# Autodesk Inventor assembly: servoAssembly
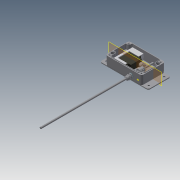
[picture p0: Inventor's stored thumbnail of the model, 180x180]
Saved by Autodesk Inventor 2018 (Build 220112000, 112)
## iProperties
Created: 2020-02-20
Part Number: servoAssembly
Document SubType Name: Assembly
Designer: anirudh
Author: anirudh
## Documents named in this file (10)
- D:\Silicon Sharks\2019-2020\servoBox\servoAssembly.iam
- D:\Silicon Sharks\2019-2020\servoBox\gripperServo.ipt
- D:\Silicon Sharks\2019-2020\servoBox\box5\AN-12B_AN-12BF-01.ipt
- D:\Silicon Sharks\2019-2020\servoBox\615438 assembly.ipt
- D:\Silicon Sharks\2019-2020\servoBox\box5\AN-12C_AN-12C-01.ipt
- D:\Silicon Sharks\2019-2020\servoBox\shaftSeal\8183K600_SUBMERSIBLE LIQUID-TIGHT CORD GRIP.ipt
- D:\Silicon Sharks\2019-2020\servoBox\shaftSeal\cordGripGasket.ipt
- D:\Silicon Sharks\2019-2020\servoBox\shaftSeal\1257K530_MINIATURE 303 STAINLESS STEEL DRIVE SHAFT.ipt
- D:\Silicon Sharks\2019-2020\servoBox\6462K190_SET SCREW SHAFT COLLAR.ipt
- D:\Silicon Sharks\2019-2020\servoBox\servoMount.ipt
## Components (10 placed, 9 different names)
1. gripperServo:1 — Mate:3, Mate:4, Mate:5, Flush:3
2. AN-12B_AN-12BF-01:1 — Mate:5, Mate:7, Mate:8, Mate:9, Mate:10, Mate:11, Mate:14, Flush:3, Mate:18, Mate:19, Mate:20
3. 615438 assembly:2 — Mate:3, Mate:4
4. AN-12C_AN-12C-01:1 — Mate:7, Mate:8, Mate:9
5. 8183K600_SUBMERSIBLE LIQUID-TIGHT CORD GRIP:1 — Mate:12, Flush:1, Flush:2, Mate:13
6. cordGripGasket:1 — Mate:10, Mate:11, Mate:12, Flush:1, Flush:2
7. 1257K530_MINIATURE 303 STAINLESS STEEL DRIVE SHAFT:1 — Mate:13, Mate:14, Mate:15, Mate:16
8. 6462K190_SET SCREW SHAFT COLLAR:1 — Mate:16, Mate:17
9. 615438 assembly:3 — Mate:15, Mate:17
10. servoMount:1 — Mate:18, Mate:19, Mate:20
## Relationships (20: Mate 17, Flush 3)
- Mate:3: gripperServo:1 ↔ 615438 assembly:2
- Mate:4: gripperServo:1 ↔ 615438 assembly:2
- Mate:5: gripperServo:1 ↔ AN-12B_AN-12BF-01:1
- Mate:7: AN-12B_AN-12BF-01:1 ↔ AN-12C_AN-12C-01:1
- Mate:8: AN-12B_AN-12BF-01:1 ↔ AN-12C_AN-12C-01:1
- Mate:9: AN-12B_AN-12BF-01:1 ↔ AN-12C_AN-12C-01:1
- Mate:10: AN-12B_AN-12BF-01:1 ↔ cordGripGasket:1
- Mate:11: AN-12B_AN-12BF-01:1 ↔ cordGripGasket:1
- Mate:12: 8183K600_SUBMERSIBLE LIQUID-TIGHT CORD GRIP:1 ↔ cordGripGasket:1
- Flush:1: 8183K600_SUBMERSIBLE LIQUID-TIGHT CORD GRIP:1 ↔ cordGripGasket:1
- Flush:2: 8183K600_SUBMERSIBLE LIQUID-TIGHT CORD GRIP:1 ↔ cordGripGasket:1
- Mate:13: 8183K600_SUBMERSIBLE LIQUID-TIGHT CORD GRIP:1 ↔ 1257K530_MINIATURE 303 STAINLESS STEEL DRIVE SHAFT:1
- Mate:14 (-27.94 mm): AN-12B_AN-12BF-01:1 ↔ 1257K530_MINIATURE 303 STAINLESS STEEL DRIVE SHAFT:1
- Mate:15: 1257K530_MINIATURE 303 STAINLESS STEEL DRIVE SHAFT:1 ↔ 615438 assembly:3
- Mate:16: 1257K530_MINIATURE 303 STAINLESS STEEL DRIVE SHAFT:1 ↔ 6462K190_SET SCREW SHAFT COLLAR:1
- Mate:17: 6462K190_SET SCREW SHAFT COLLAR:1 ↔ 615438 assembly:3
- Flush:3: gripperServo:1 ↔ AN-12B_AN-12BF-01:1
- Mate:18: AN-12B_AN-12BF-01:1 ↔ servoMount:1
- Mate:19: AN-12B_AN-12BF-01:1 ↔ servoMount:1
- Mate:20: AN-12B_AN-12BF-01:1 ↔ servoMount:1
